# Autodesk Inventor assembly: Sestava
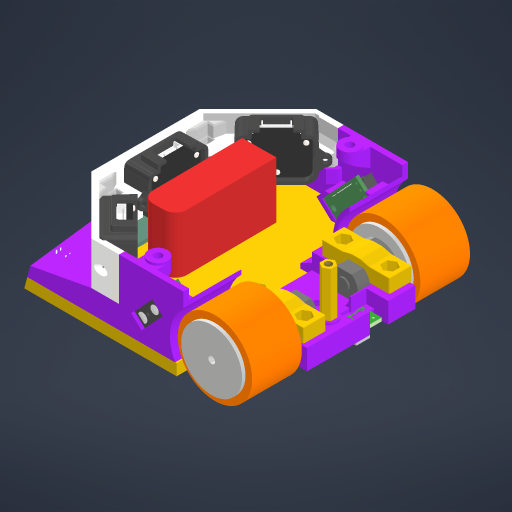
[picture p0: Inventor's stored thumbnail of the model, 512x512]
Saved by Autodesk Inventor 2024 (Build 280153000, 153)
## iProperties
Created: 2024-01-31
Part Number: Sestava
Document SubType Name: Assembly
Designer: Simak
Author: Simak
## Documents named in this file (15)
- C:\Users\Simak\OneDrive\Dokumenty\GitHub\RoboCop\- 3D -\_wip\Sestava.iam
- C:\Users\Simak\OneDrive\Dokumenty\GitHub\RoboCop\- 3D -\mech._parts\base_plate_v2.ipt
- C:\Users\Simak\OneDrive\Dokumenty\GitHub\RoboCop\- 3D -\PCBs\QRE MiniBoards\QRE MiniBoards\QRE_MiniBoards_Board.iam
- C:\Users\Simak\OneDrive\Dokumenty\GitHub\RoboCop\- 3D -\_wip\body.ipt
- C:\Users\Simak\OneDrive\Dokumenty\GitHub\RoboCop\- 3D -\mech._parts\box.ipt
- C:\Users\Simak\OneDrive\Dokumenty\GitHub\RoboCop\- 3D -\mech._parts\JSUMO_Wheel_33x25mm.ipt
- C:\Users\Simak\OneDrive\Dokumenty\GitHub\RoboCop\- 3D -\el._parts\3s lipo.ipt
- C:\Users\Simak\OneDrive\Dokumenty\GitHub\RoboCop\- 3D -\el._parts\2s lipo.ipt
- C:\Users\Simak\OneDrive\Dokumenty\GitHub\RoboCop\- 3D -\mech._parts\m3x20mm distanční sloupek.ipt
- C:\Users\Simak\OneDrive\Dokumenty\GitHub\RoboCop\- 3D -\el._parts\GA12-N20_Motor.ipt
- C:\Users\Simak\OneDrive\Dokumenty\GitHub\RoboCop\- 3D -\mech._parts\motor_C_clamp_nutt_motor_otoceny.ipt
- C:\Users\Simak\OneDrive\Dokumenty\GitHub\RoboCop\- 3D -\_wip\TF-Luna_holder_v2\TF-Luna_holder_sestava_v2.iam
- C:\Users\Simak\OneDrive\Dokumenty\GitHub\RoboCop\- 3D -\el._parts\SensorSharpDigital\side_senzor.iam
- C:\Users\Simak\OneDrive\Dokumenty\GitHub\RoboCop\- 3D -\el._parts\qre_module_V2.ipt
- C:\Users\Simak\OneDrive\Dokumenty\GitHub\RoboCop\- 3D -\PCBs\main board\sumec.iam
## Components (18 placed, 14 different names)
1. base_plate_v2:1 — Proti sobě:3, Stejný směr:2, Vložit:1, Proti sobě:4, Stejný směr:3, Stejný směr:4, Proti sobě:7, Proti sobě:8, Proti sobě:9
2. QRE_MiniBoards_Board:1 [sub-assembly] — Proti sobě:3, Stejný směr:2, Vložit:1
3. body:1 — Proti sobě:4, Stejný směr:3, Stejný směr:4, Stejný směr:5, Stejný směr:6, Proti sobě:17, Proti sobě:18, Proti sobě:20, Vložit:3, Stejný směr:7, Proti sobě:25, Proti sobě:26, Stejný směr:9, Stejný směr:10, Vložit:4, Vložit:6, Proti sobě:27, Vložit:7, Proti sobě:28, Vložit:8, Vložit:9, Stejný směr:13, Stejný směr:14
4. box:1 — Proti sobě:7, Proti sobě:8, Proti sobě:9, Proti sobě:10, Tečnost:1, Tečnost:2
5. JSUMO_Wheel_33x25mm:1 — Stejný směr:5, Proti sobě:11, Proti sobě:16
6. JSUMO_Wheel_33x25mm:2 — Proti sobě:10, Tečnost:1, Tečnost:2, Proti sobě:11, Proti sobě:19
7. 3s lipo:1
8. 2s lipo:1
9. m3x20mm distanční sloupek:1 — Stejný směr:6, Stejný směr:10, Vložit:4
10. GA12-N20_Motor:1 — Proti sobě:16, Proti sobě:17, Proti sobě:18, Proti sobě:21, Proti sobě:22
11. GA12-N20_Motor:2 — Proti sobě:19, Proti sobě:20, Proti sobě:21, Proti sobě:23
12. motor_C_clamp_nutt_motor_otoceny:1 — Proti sobě:22, Vložit:3, Stejný směr:7, Stejný směr:8, Proti sobě:24
13. motor_C_clamp_nutt_motor_otoceny:2 — Proti sobě:23, Stejný směr:8, Proti sobě:24
14. TF-Luna_holder_sestava_v2:1 [sub-assembly] — Proti sobě:25, Proti sobě:26, Stejný směr:9
15. side_senzor:1 [sub-assembly] — Vložit:6, Proti sobě:27
16. side_senzor:2 [sub-assembly] — Vložit:7, Proti sobě:28
17. qre_module_V2:1 — Vložit:8, Stejný směr:14
18. sumec:1 [sub-assembly] — Vložit:9, Stejný směr:13
## Relationships (40: Mate 20, Flush 11, Insert 7, Tangent 2)
- Proti sobě:3 [Mate] (1 mm): base_plate_v2:1 ↔ QRE_MiniBoards_Board:1
- Stejný směr:2 [Flush] (4.75 mm): base_plate_v2:1 ↔ QRE_MiniBoards_Board:1
- Vložit:1 [Insert]: base_plate_v2:1 ↔ QRE_MiniBoards_Board:1
- Proti sobě:4 [Mate]: base_plate_v2:1 ↔ body:1
- Stejný směr:3 [Flush]: base_plate_v2:1 ↔ body:1
- Stejný směr:4 [Flush]: base_plate_v2:1 ↔ body:1
- Proti sobě:7 [Mate] (2.5 mm): base_plate_v2:1 ↔ box:1
- Proti sobě:8 [Mate]: base_plate_v2:1 ↔ box:1
- Proti sobě:9 [Mate]: base_plate_v2:1 ↔ box:1
- Proti sobě:10 [Mate]: box:1 ↔ JSUMO_Wheel_33x25mm:2
- Tečnost:1 [Tangent]: box:1 ↔ JSUMO_Wheel_33x25mm:2
- Tečnost:2 [Tangent]: box:1 ↔ JSUMO_Wheel_33x25mm:2
- Stejný směr:5 [Flush]: body:1 ↔ JSUMO_Wheel_33x25mm:1
- Proti sobě:11 [Mate]: JSUMO_Wheel_33x25mm:1 ↔ JSUMO_Wheel_33x25mm:2
- Stejný směr:6 [Flush]: body:1 ↔ m3x20mm distanční sloupek:1
- Proti sobě:16 [Mate]: JSUMO_Wheel_33x25mm:1 ↔ GA12-N20_Motor:1
- Proti sobě:17 [Mate]: body:1 ↔ GA12-N20_Motor:1
- Proti sobě:18 [Mate]: body:1 ↔ GA12-N20_Motor:1
- Proti sobě:19 [Mate]: JSUMO_Wheel_33x25mm:2 ↔ GA12-N20_Motor:2
- Proti sobě:20 [Mate]: body:1 ↔ GA12-N20_Motor:2
- Proti sobě:21 [Mate] (18 mm): GA12-N20_Motor:1 ↔ GA12-N20_Motor:2
- Proti sobě:22 [Mate]: GA12-N20_Motor:1 ↔ motor_C_clamp_nutt_motor_otoceny:1
- Vložit:3 [Insert]: body:1 ↔ motor_C_clamp_nutt_motor_otoceny:1
- Stejný směr:7 [Flush]: body:1 ↔ motor_C_clamp_nutt_motor_otoceny:1
- Proti sobě:23 [Mate]: GA12-N20_Motor:2 ↔ motor_C_clamp_nutt_motor_otoceny:2
- Stejný směr:8 [Flush]: motor_C_clamp_nutt_motor_otoceny:1 ↔ motor_C_clamp_nutt_motor_otoceny:2
- Proti sobě:24 [Mate] (28 mm): motor_C_clamp_nutt_motor_otoceny:1 ↔ motor_C_clamp_nutt_motor_otoceny:2
- Proti sobě:25 [Mate]: body:1 ↔ TF-Luna_holder_sestava_v2:1
- Proti sobě:26 [Mate]: body:1 ↔ TF-Luna_holder_sestava_v2:1
- Stejný směr:9 [Flush]: body:1 ↔ TF-Luna_holder_sestava_v2:1
- Stejný směr:10 [Flush]: body:1 ↔ m3x20mm distanční sloupek:1
- Vložit:4 [Insert]: body:1 ↔ m3x20mm distanční sloupek:1
- Vložit:6 [Insert]: body:1 ↔ side_senzor:1
- Proti sobě:27 [Mate]: body:1 ↔ side_senzor:1
- Vložit:7 [Insert]: body:1 ↔ side_senzor:2
- Proti sobě:28 [Mate]: body:1 ↔ side_senzor:2
- Vložit:8 [Insert]: body:1 ↔ qre_module_V2:1
- Vložit:9 [Insert]: body:1 ↔ sumec:1
- Stejný směr:13 [Flush]: body:1 ↔ sumec:1
- Stejný směr:14 [Flush]: body:1 ↔ qre_module_V2:1
## Named parameters: Finish1_Area = 2.15
note: some values were not read from the file. Shown as the stored number, unit unknown: "Finish1_Area".
